# Autodesk Inventor assembly: Servo Assembly
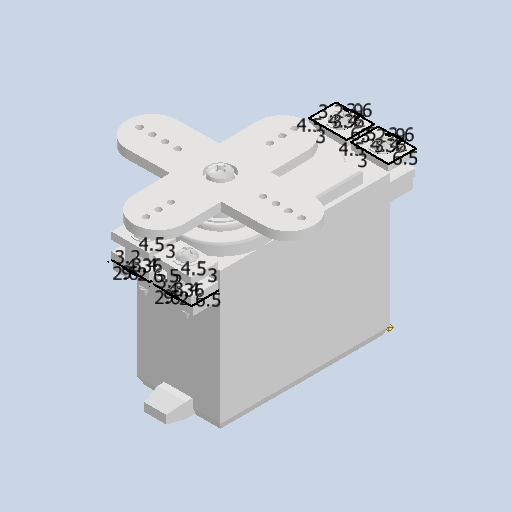
[picture p0: Inventor's stored thumbnail of the model, 512x512]
Saved by Autodesk Inventor 2023 (Build 270158000, 158)
## iProperties
Created: 2023-09-05
Part Number: Servo Assembly
Document SubType Name: Assembly
Designer: Nate
Author: Nate
## Documents named in this file (7)
- C:\Users\Nate\Documents\CAD_Assignment_2\Servo Assembly\Servo Assembly.iam
- C:\Users\Nate\Documents\CAD_Assignment_2\Parts\Hitec HS-425BB Servo.ipt
- C:\Users\Nate\Documents\CAD_Assignment_2\Parts\Standard Servo Rubber Grommet.ipt
- C:\Users\Nate\Documents\CAD_Assignment_2\Parts\Standard Servo Brass Sleeve.ipt
- C:\Users\Nate\Documents\CAD_Assignment_2\Parts\Standar Servo Horn - Red.ipt
- C:\Users\Nate\Documents\CAD_Assignment_2\McMaster-Carr imports\90184A064_Phillips Rounded Head Screws for Sheet Metal.ipt
- C:\Users\Nate\Documents\CAD_Assignment_2\McMaster-Carr imports\95836A255_Black-Oxide 18-8 Stainless Steel Pan Head Phillips Screws.ipt
## Components (15 placed, 6 different names)
1. Hitec HS-425BB Servo:1 — Insert:1, Insert:2, Insert:3, Insert:4, Insert:9
2. Standard Servo Rubber Grommet:1 — Insert:1, Insert:6
3. Standard Servo Rubber Grommet:2 — Insert:2, Insert:5
4. Standard Servo Rubber Grommet:3 — Insert:3, Insert:8
5. Standard Servo Rubber Grommet:4 — Insert:4, Insert:7
6. Standard Servo Brass Sleeve:1 — Insert:6, Insert:13
7. Standard Servo Brass Sleeve:2 — Insert:7, Insert:10
8. Standard Servo Brass Sleeve:3 — Insert:5, Insert:14
9. Standard Servo Brass Sleeve:4 — Insert:8, Insert:11
10. Standar Servo Horn - Red:1 — Insert:9, Insert:12
11. 90184A064_Phillips Rounded Head Screws for Sheet Metal:1 — Insert:13
12. 90184A064_Phillips Rounded Head Screws for Sheet Metal:2 — Insert:11
13. 90184A064_Phillips Rounded Head Screws for Sheet Metal:3 — Insert:14
14. 90184A064_Phillips Rounded Head Screws for Sheet Metal:4 — Insert:10
15. 95836A255_Black-Oxide 18-8 Stainless Steel Pan Head Phillips Screws:1 — Insert:12
## Relationships (14: Insert 14)
- Insert:1: Hitec HS-425BB Servo:1 ↔ Standard Servo Rubber Grommet:1
- Insert:2: Hitec HS-425BB Servo:1 ↔ Standard Servo Rubber Grommet:2
- Insert:3: Hitec HS-425BB Servo:1 ↔ Standard Servo Rubber Grommet:3
- Insert:4: Hitec HS-425BB Servo:1 ↔ Standard Servo Rubber Grommet:4
- Insert:5: Standard Servo Rubber Grommet:2 ↔ Standard Servo Brass Sleeve:3
- Insert:6: Standard Servo Rubber Grommet:1 ↔ Standard Servo Brass Sleeve:1
- Insert:7: Standard Servo Rubber Grommet:4 ↔ Standard Servo Brass Sleeve:2
- Insert:8: Standard Servo Rubber Grommet:3 ↔ Standard Servo Brass Sleeve:4
- Insert:9: Hitec HS-425BB Servo:1 ↔ Standar Servo Horn - Red:1
- Insert:10: Standard Servo Brass Sleeve:2 ↔ 90184A064_Phillips Rounded Head Screws for Sheet Metal:4
- Insert:11: Standard Servo Brass Sleeve:4 ↔ 90184A064_Phillips Rounded Head Screws for Sheet Metal:2
- Insert:12: Standar Servo Horn - Red:1 ↔ 95836A255_Black-Oxide 18-8 Stainless Steel Pan Head Phillips Screws:1
- Insert:13: Standard Servo Brass Sleeve:1 ↔ 90184A064_Phillips Rounded Head Screws for Sheet Metal:1
- Insert:14: Standard Servo Brass Sleeve:3 ↔ 90184A064_Phillips Rounded Head Screws for Sheet Metal:3
